# Autodesk Inventor assembly: Drive Base Assembly
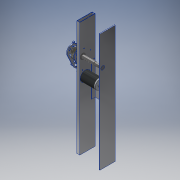
[picture p0: Inventor's stored thumbnail of the model, 180x180]
Saved by Autodesk Inventor 2019.4 (Build 234330000, 330)
## iProperties
Created: 2019-11-02
Part Number: Drive Base Assembly
Document SubType Name: Assembly
Designer: admin
Author: admin
## Documents named in this file (16)
- C:\Users\admin\Desktop\FRC 2020 Engineering\GitHub\7738-CAD-prep\Butterfly Drive Mk2\Butterfly Base\Drive Base Assembly.iam
- C:\Users\admin\Desktop\FRC 2020 Engineering\GitHub\7738-CAD-prep\Butterfly Drive Mk2\Butterfly Base\Main Axle.ipt
- C:\Users\admin\Desktop\FRC 2020 Engineering\GitHub\7738-CAD-prep\Butterfly Drive Mk2\Butterfly Module\Butterfly Drive Module.iam
- C:\Users\admin\Desktop\FRC 2020 Engineering\GitHub\7738-CAD-prep\Butterfly Drive Mk2\Butterfly Base\Side Extrusion.ipt
- C:\Users\admin\Desktop\FRC 2020 Engineering\GitHub\7738-CAD-prep\am-0255 2.5inch CIM Motor.ipt
- C:\Users\admin\Desktop\FRC 2020 Engineering\GitHub\7738-CAD-prep\Butterfly Drive Mk2\Butterfly Base\Mottor Protection Piece.ipt
- C:\Users\admin\Desktop\FRC 2020 Engineering\GitHub\7738-CAD-prep\Butterfly Drive Mk2\Butterfly Base\Drive Base Assembly\Design Accelerator\Spur Gears1.iam
- C:\Users\admin\Desktop\FRC 2020 Engineering\GitHub\7738-CAD-prep\Butterfly Drive Mk2\Butterfly Base\Drive Base Assembly\Design Accelerator\Spur Gears2.iam
- C:\Users\admin\Desktop\FRC 2020 Engineering\GitHub\7738-CAD-prep\Butterfly Drive Mk2\Butterfly Base\Drive Base Assembly\Design Accelerator\Spur Gears3.iam
- C:\Users\admin\Desktop\FRC 2020 Engineering\GitHub\7738-CAD-prep\Butterfly Drive Mk2\Butterfly Base\F6004.ipt
- C:\Users\admin\Desktop\FRC 2020 Engineering\GitHub\7738-CAD-prep\Butterfly Drive Mk2\Butterfly Base\F6802.ipt
- C:\Users\admin\Desktop\FRC 2020 Engineering\GitHub\7738-CAD-prep\Butterfly Drive Mk2\Butterfly Base\F6800Z 10mm ID Flange.ipt
- C:\Users\admin\Desktop\FRC 2020 Engineering\GitHub\7738-CAD-prep\Butterfly Drive Mk2\Butterfly Base\Gearbob Plate.ipt
- C:\Users\admin\Desktop\FRC 2020 Engineering\GitHub\7738-CAD-prep\Butterfly Drive Mk2\Butterfly Base\Gearbob Plate 3mm.ipt
- C:\Users\admin\Desktop\FRC 2020 Engineering\GitHub\7738-CAD-prep\Butterfly Drive Mk2\Butterfly Base\Bumper Plate.ipt
- C:\Users\admin\Desktop\FRC 2020 Engineering\GitHub\7738-CAD-prep\Butterfly Drive Mk2\Butterfly Base\Gearbox Axle 1.ipt
## Components (21 placed, 13 different names)
1. Main Axle:1 — Mate:28, Mate:29, Mate:40, Mate:49, Mate:52
2. Butterfly Drive Module:1 [sub-assembly] — Mate:2, Mate:7, Mate:40, Mate:48
3. Side Extrusion:1 — Mate:2, Mate:5, Flush:2, Mate:8, Mate:10, Flush:3, Flush:4, Mate:17, Mate:19, Angle:2, Mate:43, Flush:6, Mate:44, Mate:45, Mate:46, Mate:47, Flush:7, Flush:8, Mate:53
4. am-0255 2.5inch CIM Motor:1 — Mate:12, Mate:17, Mate:19, Mate:43, Mate:44
5. Motor Protection Piece:1 — Mate:5, Flush:2, Flush:6
6. Spur Gears:1 [sub-assembly] — Mate:11, Mate:14, Mate:16, Mate:18, Mate:20, Mate:21, Mate:35, Mate:41, Mate:42
7. Spur Gears:2 [sub-assembly] — Mate:7, Mate:8, Mate:11, Mate:18
8. Spur Gears:3 [sub-assembly] — Mate:12, Mate:14, Mate:16
9. F6802:1 — Mate:51, Mate:56
10. F6800Z 10mm ID Flange:1 — Mate:28, Mate:29, Flush:5, Mate:39
11. F6800Z 10mm ID Flange:2 — Mate:35, Flush:5, Mate:38, Mate:57, Flush:9
12. Gearbob Plate:1 — Mate:38, Mate:39, Mate:41, Mate:42, Mate:60, Mate:61
13. Gearbob Plate 3mm:1 — Mate:45, Mate:46, Mate:47, Mate:51, Mate:54, Mate:55, Mate:56, Mate:58, Mate:59
14. Bumper Plate:1 — Flush:7, Flush:8, Mate:48, Mate:50
15. F6802:2 — Mate:49, Mate:50
16. F6004:2 — Mate:52, Mate:53
17. F6800Z 10mm ID Flange:3 — Mate:54, Mate:55
18. Gearbox Axle 1:1 — Mate:57, Flush:9
19. F6800Z 10mm ID Flange:4 — Mate:58, Mate:59
20. F6800Z 10mm ID Flange:5 — Mate:60, Mate:61, Mate:62, Flush:10
21. Gearbox Axle 1:2 — Mate:62, Flush:10
## Relationships (52: Mate 42, Flush 9, Angle 1)
- Mate:2 (6.5 mm): Butterfly Drive Module:1 ↔ Side Extrusion:1
- Mate:5 (0.5 mm): Side Extrusion:1 ↔ Motor Protection Piece:1
- Flush:2: Side Extrusion:1 ↔ Motor Protection Piece:1
- Mate:7: Butterfly Drive Module:1 ↔ Spur Gears:2
- Mate:8 (7 mm): Side Extrusion:1 ↔ Spur Gears:2
- Mate:10: Side Extrusion:1
- Flush:3: Side Extrusion:1
- Flush:4: Side Extrusion:1
- Mate:11 (5 mm): Spur Gears:1 ↔ Spur Gears:2
- Mate:12: am-0255 2.5inch CIM Motor:1 ↔ Spur Gears:3
- Mate:14 (5 mm): Spur Gears:1 ↔ Spur Gears:3
- Mate:16: Spur Gears:1 ↔ Spur Gears:3
- Mate:17 (0.3 mm): Side Extrusion:1 ↔ am-0255 2.5inch CIM Motor:1
- Mate:18: Spur Gears:1 ↔ Spur Gears:2
- Mate:19: Side Extrusion:1 ↔ am-0255 2.5inch CIM Motor:1
- Mate:20: Spur Gears:1
- Mate:21: Spur Gears:1
- Angle:2 (0 deg): Side Extrusion:1
- Mate:28: Main Axle:1 ↔ F6800Z 10mm ID Flange:1
- Mate:29 (0.3 mm): Main Axle:1 ↔ F6800Z 10mm ID Flange:1
- Mate:35: Spur Gears:1 ↔ F6800Z 10mm ID Flange:2
- Flush:5: F6800Z 10mm ID Flange:1 ↔ F6800Z 10mm ID Flange:2
- Mate:38: F6800Z 10mm ID Flange:2 ↔ Gearbob Plate:1
- Mate:39 (0.3 mm): F6800Z 10mm ID Flange:1 ↔ Gearbob Plate:1
- Mate:40: Main Axle:1 ↔ Butterfly Drive Module:1
- Mate:41 (4 mm): Spur Gears:1 ↔ Gearbob Plate:1
- Mate:42: Spur Gears:1 ↔ Gearbob Plate:1
- Mate:43: Side Extrusion:1 ↔ am-0255 2.5inch CIM Motor:1
- Flush:6 (270 mm): Side Extrusion:1 ↔ Motor Protection Piece:1
- Mate:44: Side Extrusion:1 ↔ am-0255 2.5inch CIM Motor:1
- Mate:45: Side Extrusion:1 ↔ Gearbob Plate 3mm:1
- Mate:46: Side Extrusion:1 ↔ Gearbob Plate 3mm:1
- Mate:47 (0.2 mm): Side Extrusion:1 ↔ Gearbob Plate 3mm:1
- Flush:7: Side Extrusion:1 ↔ Bumper Plate:1
- Flush:8: Side Extrusion:1 ↔ Bumper Plate:1
- Mate:48 (6.5 mm): Butterfly Drive Module:1 ↔ Bumper Plate:1
- Mate:49: Main Axle:1 ↔ F6802:2
- Mate:50 (0.3 mm): Bumper Plate:1 ↔ F6802:2
- Mate:51 (0.3 mm): F6802:1 ↔ Gearbob Plate 3mm:1
- Mate:52: Main Axle:1 ↔ F6004:2
- Mate:53 (0.3 mm): Side Extrusion:1 ↔ F6004:2
- Mate:54: Gearbob Plate 3mm:1 ↔ F6800Z 10mm ID Flange:3
- Mate:55 (0.3 mm): Gearbob Plate 3mm:1 ↔ F6800Z 10mm ID Flange:3
- Mate:56: F6802:1 ↔ Gearbob Plate 3mm:1
- Mate:57: F6800Z 10mm ID Flange:2 ↔ Gearbox Axle 1:1
- Flush:9: F6800Z 10mm ID Flange:2 ↔ Gearbox Axle 1:1
- Mate:58: Gearbob Plate 3mm:1 ↔ F6800Z 10mm ID Flange:4
- Mate:59 (0.3 mm): Gearbob Plate 3mm:1 ↔ F6800Z 10mm ID Flange:4
- Mate:60 (0.3 mm): Gearbob Plate:1 ↔ F6800Z 10mm ID Flange:5
- Mate:61: Gearbob Plate:1 ↔ F6800Z 10mm ID Flange:5
- Mate:62: F6800Z 10mm ID Flange:5 ↔ Gearbox Axle 1:2
- Flush:10: F6800Z 10mm ID Flange:5 ↔ Gearbox Axle 1:2
